# Autodesk Inventor assembly: Single Header Pin
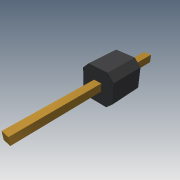
[picture p0: Inventor's stored thumbnail of the model, 180x180]
Saved by Autodesk Inventor 2016 (Build 200138000, 138)
## iProperties
Created: 2016-01-25
Part Number: Single Header Pin
Document SubType Name: Assembly
Designer: larraguetajunior
Author: larraguetajunior
## Documents named in this file (3)
- D:\cloud\Dropbox\UAV\- Air Data Computer\Asgard\Off the shelf\teensy3.6\Single Header Pin.iam
- D:\cloud\Dropbox\UAV\- Air Data Computer\Asgard\Off the shelf\teensy3.6\Straight Header Pin.ipt
- D:\cloud\Dropbox\UAV\- Air Data Computer\Asgard\Off the shelf\teensy3.6\Pin Stopper 0.6mm.ipt
## Components (2 placed, 2 different names)
1. Straight Header Pin:1 — Mate:1, Mate:2, Flush:1, Mate:3, Mate:4, Flush:2
2. Pin Stopper 0.6mm:1 — Mate:3, Mate:4, Flush:2
## Relationships (6: Mate 4, Flush 2)
- Mate:1: Straight Header Pin:1
- Mate:2: Straight Header Pin:1
- Flush:1: Straight Header Pin:1
- Mate:3: Straight Header Pin:1 ↔ Pin Stopper 0.6mm:1
- Mate:4: Straight Header Pin:1 ↔ Pin Stopper 0.6mm:1
- Flush:2 (2.6 mm): Straight Header Pin:1 ↔ Pin Stopper 0.6mm:1
